# Autodesk Inventor assembly: Main Assembly
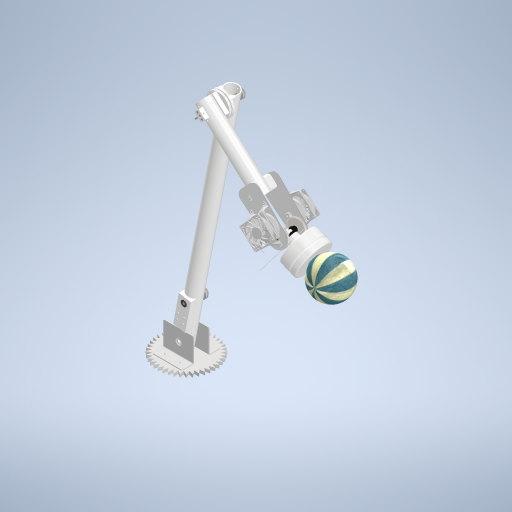
[picture p0: Inventor's stored thumbnail of the model, 512x512]
Saved by Autodesk Inventor 2023 (Build 270158000, 158)
## iProperties
Created: 2022-10-01
Part Number: Main Assembly
Document SubType Name: Assembly
Designer: cjj5381
Mass: 5668.97 g
Surface Area: 15277.1 cm^2
Volume: 4706.26 cm^3
Density: 1.20456 g/cm^3
Author: cjj5381
## Documents named in this file (24)
- C:\Users\t205b\OneDrive\Documents\Github\BehrendURCMechanical\CAD\Apparatus\THE ARM\Main Assembly.iam
- C:\Users\t205b\OneDrive\Documents\Github\BehrendURCMechanical\CAD\Apparatus\THE ARM\Arm Segment 1.ipt
- C:\Users\t205b\OneDrive\Documents\Github\BehrendURCMechanical\CAD\Apparatus\THE ARM\3 Stage HD - CIM Sport.iam
- C:\Users\t205b\OneDrive\Documents\Github\BehrendURCMechanical\CAD\Apparatus\THE ARM\Arm Segment 2.ipt
- C:\Users\t205b\OneDrive\Documents\Github\BehrendURCMechanical\CAD\Apparatus\THE ARM\Wrist\Wrist.iam
- C:\Users\t205b\OneDrive\Documents\Github\BehrendURCMechanical\CAD\Apparatus\THE ARM\Versaball.iam
- C:\Users\t205b\OneDrive\Documents\Github\BehrendURCMechanical\CAD\Apparatus\THE ARM\Hardware\91290A224_NO THREADS_Alloy Steel Socket Head Screw.ipt
- C:\Users\t205b\OneDrive\Documents\Github\BehrendURCMechanical\CAD\Apparatus\THE ARM\Hub Plate.ipt
- C:\Users\t205b\OneDrive\Documents\Github\BehrendURCMechanical\CAD\Apparatus\THE ARM\Hardware\5909K15_Needle-Roller Thrust Bearing.ipt
- C:\Users\t205b\OneDrive\Documents\Github\BehrendURCMechanical\CAD\Apparatus\THE ARM\Hardware\5909K75_1 mm Thick Washer for 20 mm Shaft Diameter Needle-Roller Thrust Bearing.ipt
- C:\Users\t205b\OneDrive\Documents\Github\BehrendURCMechanical\CAD\Apparatus\THE ARM\Motor Mount.ipt
- C:\Users\t205b\OneDrive\Documents\Github\BehrendURCMechanical\CAD\Apparatus\THE ARM\Hardware\91251A342_NO THREADS_Black-Oxide Alloy Steel Socket Head Screw.ipt
- C:\Users\t205b\OneDrive\Documents\Github\BehrendURCMechanical\CAD\Apparatus\THE ARM\Hardware\1265K77_Rotary Shaft-longer.ipt
- C:\Users\t205b\OneDrive\Documents\Github\BehrendURCMechanical\CAD\Apparatus\THE ARM\Axial Holder.ipt
- C:\Users\t205b\OneDrive\Documents\Github\BehrendURCMechanical\CAD\Apparatus\THE ARM\Hardware\GPA60GT2060-B-NK10.iam
- C:\Users\t205b\OneDrive\Documents\Github\BehrendURCMechanical\CAD\Apparatus\THE ARM\Hardware\2349K412_Permanently Lubricated Ball Bearing.ipt
- C:\Users\t205b\OneDrive\Documents\Github\BehrendURCMechanical\CAD\Apparatus\THE ARM\Hardware\1265K77_Rotary Shaft short.ipt
- C:\Users\t205b\OneDrive\Documents\Github\BehrendURCMechanical\CAD\Apparatus\THE ARM\Base\Base.iam
- C:\Users\t205b\OneDrive\Documents\Github\BehrendURCMechanical\CAD\Apparatus\THE ARM\Hardware\94645A102_NO THREADS_High-Strength Steel Nylon-Insert Locknut.ipt
- C:\Users\t205b\OneDrive\Documents\Github\BehrendURCMechanical\CAD\Apparatus\THE ARM\Hardware\94180A361_NO THREADS_Tapered Heat-Set Inserts for Plastic.ipt
- C:\Users\t205b\OneDrive\Documents\Github\BehrendURCMechanical\CAD\Apparatus\THE ARM\Hardware\91290A252_NO THREADS_Alloy Steel Socket Head Screw.ipt
- C:\Users\t205b\OneDrive\Documents\Github\BehrendURCMechanical\CAD\Apparatus\THE ARM\Hardware\91290A195_Black-Oxide Alloy Steel Socket Head Screw.ipt
- C:\Users\t205b\OneDrive\Documents\Github\BehrendURCMechanical\CAD\Apparatus\THE ARM\Hardware\91290A195_Black-Oxide Alloy Steel Socket Head Screw_CPY.ipt
- C:\Users\t205b\OneDrive\Documents\Github\BehrendURCMechanical\CAD\Apparatus\THE ARM\Hardware\1265K17_Rotary Shaft.ipt
## Components (45 placed, 23 different names)
1. Base:1 [sub-assembly] — Mate:1, Flush:1, Mate:2, Mate:3
2. Arm Segment 1:1 — Mate:2, Mate:3, Mate:4, Mate:5, Mate:12, Mate:13, Mate:48, Mate:49, Mate:50, Mate:51
3. 3 Stage HD - CIM Sport:2 [sub-assembly]
4. Arm Segment 2:1 — Mate:20, Mate:21, Mate:22, Mate:23, Mate:44, Mate:45, Mate:46, Mate:47, Mate:52, Flush:11
5. Wrist:1 [sub-assembly] — Mate:52, Flush:11, Mate:54, Mate:55, Mate:56, Mate:57, Mate:58, Mate:59, Mate:60, Mate:61, Mate:62, Mate:63
6. Versaball:1 [sub-assembly] — Mate:54, Mate:55, Mate:68
7. Hub Plate:1 — Mate:18, Mate:19, Mate:20, Mate:21, Mate:39, Mate:40, Mate:41, Flush:8
8. Hub Plate:2 — Mate:12, Mate:13, Mate:16, Mate:17, Mate:18, Mate:42, Flush:9, Mate:43, Flush:10
9. 5909K15_Needle-Roller Thrust Bearing:1 — Mate:14, Tangent:1, Tangent:2, Mate:15
10. 5909K75_1 mm Thick Washer for 20 mm Shaft Diameter Needle-Roller Thrust Bearing:1 — Mate:14, Tangent:1, Mate:17
11. 5909K75_1 mm Thick Washer for 20 mm Shaft Diameter Needle-Roller Thrust Bearing:2 — Tangent:2, Mate:15, Mate:16, Mate:19
12. Motor Mount:1 — Mate:4, Mate:5, Mate:6, Mate:7, Mate:8, Flush:2, Mate:9
13. 1265K77_Rotary Shaft-longer:1 — Mate:24, Mate:25, Mate:28, Flush:5
14. Axial Holder:1 — Mate:22, Mate:23, Mate:24, Mate:25
15. 91290A252_NO THREADS_Alloy Steel Socket Head Screw:1
16. GPA60GT2060-B-NK10:1 [sub-assembly] — Mate:28, Flush:5
17. GPA60GT2060-B-NK10:2 [sub-assembly] — Mate:11, Flush:4
18. 2349K412_Permanently Lubricated Ball Bearing:1 — Flush:2, Mate:9, Mate:10, Flush:3
19. 1265K77_Rotary Shaft short:1 — Mate:10, Flush:3, Mate:11, Flush:4
20. 3 Stage HD - CIM Sport:3 [sub-assembly]
21. 91290A252_NO THREADS_Alloy Steel Socket Head Screw:2
22. 91290A252_NO THREADS_Alloy Steel Socket Head Screw:3
23. 94645A102_NO THREADS_High-Strength Steel Nylon-Insert Locknut:1
24. 94645A102_NO THREADS_High-Strength Steel Nylon-Insert Locknut:2
25. 94180A361_NO THREADS_Tapered Heat-Set Inserts for Plastic:1 — Mate:39, Mate:40
26. 94180A361_NO THREADS_Tapered Heat-Set Inserts for Plastic:2 — Mate:41, Flush:8
27. 94180A361_NO THREADS_Tapered Heat-Set Inserts for Plastic:3 — Mate:43, Flush:10
28. 94180A361_NO THREADS_Tapered Heat-Set Inserts for Plastic:4 — Mate:42, Flush:9
29. 91290A224_NO THREADS_Alloy Steel Socket Head Screw:7 — Mate:44, Mate:45
30. 91290A224_NO THREADS_Alloy Steel Socket Head Screw:8 — Mate:46, Mate:47
31. 91290A224_NO THREADS_Alloy Steel Socket Head Screw:9 — Mate:50, Mate:51
32. 91290A224_NO THREADS_Alloy Steel Socket Head Screw:10 — Mate:48, Mate:49
33. 91290A195_Black-Oxide Alloy Steel Socket Head Screw:1 — Mate:56, Mate:57, Mate:66, Flush:13
34. 91290A195_Black-Oxide Alloy Steel Socket Head Screw_CPY:1 — Mate:58, Mate:59, Mate:67, Flush:14
35. 91290A195_Black-Oxide Alloy Steel Socket Head Screw:2 — Mate:60, Mate:61, Mate:64, Flush:15
36. 91290A195_Black-Oxide Alloy Steel Socket Head Screw:3 — Mate:62, Mate:63, Mate:65, Flush:12
37. 94645A102_NO THREADS_High-Strength Steel Nylon-Insert Locknut:3 — Mate:64, Flush:15
38. 94645A102_NO THREADS_High-Strength Steel Nylon-Insert Locknut:4 — Mate:65, Flush:12
39. 94645A102_NO THREADS_High-Strength Steel Nylon-Insert Locknut:5 — Mate:67, Flush:14
40. 94645A102_NO THREADS_High-Strength Steel Nylon-Insert Locknut:6 — Mate:66, Flush:13
41. 1265K17_Rotary Shaft:1 — Mate:68
42. 91251A342_NO THREADS_Black-Oxide Alloy Steel Socket Head Screw:1 — Mate:6
43. 91251A342_NO THREADS_Black-Oxide Alloy Steel Socket Head Screw:2 — Mate:7, Mate:8
44. 91251A342_NO THREADS_Black-Oxide Alloy Steel Socket Head Screw:3
45. 91251A342_NO THREADS_Black-Oxide Alloy Steel Socket Head Screw:4
## Component patterns: (4 elements, first: 91251A342_NO THREADS_Black-Oxide Alloy Steel Socket Head Screw:1)
## Relationships (80: Mate 63, Flush 15, Tangent 2)
- Mate:1: Base:1
- Flush:1: Base:1
- Mate:2: Base:1 ↔ Arm Segment 1:1
- Mate:3: Base:1 ↔ Arm Segment 1:1
- Mate:4: Arm Segment 1:1 ↔ Motor Mount:1
- Mate:5: Arm Segment 1:1 ↔ Motor Mount:1
- Mate:6: Motor Mount:1 ↔ 91251A342_NO THREADS_Black-Oxide Alloy Steel Socket Head Screw:1
- Mate:7: Motor Mount:1 ↔ 91251A342_NO THREADS_Black-Oxide Alloy Steel Socket Head Screw:2
- Mate:8: Motor Mount:1 ↔ 91251A342_NO THREADS_Black-Oxide Alloy Steel Socket Head Screw:2
- Flush:2: Motor Mount:1 ↔ 2349K412_Permanently Lubricated Ball Bearing:1
- Mate:9: Motor Mount:1 ↔ 2349K412_Permanently Lubricated Ball Bearing:1
- Mate:10: 2349K412_Permanently Lubricated Ball Bearing:1 ↔ 1265K77_Rotary Shaft short:1
- Flush:3: 2349K412_Permanently Lubricated Ball Bearing:1 ↔ 1265K77_Rotary Shaft short:1
- Mate:11: GPA60GT2060-B-NK10:2 ↔ 1265K77_Rotary Shaft short:1
- Flush:4: GPA60GT2060-B-NK10:2 ↔ 1265K77_Rotary Shaft short:1
- Mate:12: Arm Segment 1:1 ↔ Hub Plate:2
- Mate:13: Arm Segment 1:1 ↔ Hub Plate:2
- Mate:14: 5909K15_Needle-Roller Thrust Bearing:1 ↔ 5909K75_1 mm Thick Washer for 20 mm Shaft Diameter Needle-Roller Thrust Bearing:1
- Tangent:1: 5909K15_Needle-Roller Thrust Bearing:1 ↔ 5909K75_1 mm Thick Washer for 20 mm Shaft Diameter Needle-Roller Thrust Bearing:1
- Tangent:2: 5909K15_Needle-Roller Thrust Bearing:1 ↔ 5909K75_1 mm Thick Washer for 20 mm Shaft Diameter Needle-Roller Thrust Bearing:2
- Mate:15: 5909K15_Needle-Roller Thrust Bearing:1 ↔ 5909K75_1 mm Thick Washer for 20 mm Shaft Diameter Needle-Roller Thrust Bearing:2
- Mate:16: Hub Plate:2 ↔ 5909K75_1 mm Thick Washer for 20 mm Shaft Diameter Needle-Roller Thrust Bearing:2
- Mate:17: Hub Plate:2 ↔ 5909K75_1 mm Thick Washer for 20 mm Shaft Diameter Needle-Roller Thrust Bearing:1
- Mate:18: Hub Plate:1 ↔ Hub Plate:2
- Mate:19: Hub Plate:1 ↔ 5909K75_1 mm Thick Washer for 20 mm Shaft Diameter Needle-Roller Thrust Bearing:2
- Mate:20: Arm Segment 2:1 ↔ Hub Plate:1
- Mate:21: Arm Segment 2:1 ↔ Hub Plate:1
- Mate:22: Arm Segment 2:1 ↔ Axial Holder:1
- Mate:23: Arm Segment 2:1 ↔ Axial Holder:1
- Mate:24: 1265K77_Rotary Shaft-longer:1 ↔ Axial Holder:1
- Mate:25: 1265K77_Rotary Shaft-longer:1 ↔ Axial Holder:1
- [Mate]: Axial Holder:1 ↔ 91290A252_NO THREADS_Alloy Steel Socket Head Screw:1
- [Mate]: Axial Holder:1 ↔ 91290A252_NO THREADS_Alloy Steel Socket Head Screw:1
- Mate:28: 1265K77_Rotary Shaft-longer:1 ↔ GPA60GT2060-B-NK10:1
- Flush:5: 1265K77_Rotary Shaft-longer:1 ↔ GPA60GT2060-B-NK10:1
- [Mate]: Axial Holder:1 ↔ 91290A252_NO THREADS_Alloy Steel Socket Head Screw:2
- [Mate]: Axial Holder:1 ↔ 91290A252_NO THREADS_Alloy Steel Socket Head Screw:2
- [Mate]: Axial Holder:1 ↔ 91290A252_NO THREADS_Alloy Steel Socket Head Screw:3
- [Mate]: Axial Holder:1 ↔ 91290A252_NO THREADS_Alloy Steel Socket Head Screw:3
- [Mate]: 91290A252_NO THREADS_Alloy Steel Socket Head Screw:2 ↔ 94645A102_NO THREADS_High-Strength Steel Nylon-Insert Locknut:1
- [Flush]: 91290A252_NO THREADS_Alloy Steel Socket Head Screw:2 ↔ 94645A102_NO THREADS_High-Strength Steel Nylon-Insert Locknut:1
- [Mate]: 91290A252_NO THREADS_Alloy Steel Socket Head Screw:3 ↔ 94645A102_NO THREADS_High-Strength Steel Nylon-Insert Locknut:2
- [Flush]: 91290A252_NO THREADS_Alloy Steel Socket Head Screw:3 ↔ 94645A102_NO THREADS_High-Strength Steel Nylon-Insert Locknut:2
- Mate:39: Hub Plate:1 ↔ 94180A361_NO THREADS_Tapered Heat-Set Inserts for Plastic:1
- Mate:40 (1 mm): Hub Plate:1 ↔ 94180A361_NO THREADS_Tapered Heat-Set Inserts for Plastic:1
- Mate:41: Hub Plate:1 ↔ 94180A361_NO THREADS_Tapered Heat-Set Inserts for Plastic:2
- Flush:8 (-1 mm): Hub Plate:1 ↔ 94180A361_NO THREADS_Tapered Heat-Set Inserts for Plastic:2
- Mate:42: Hub Plate:2 ↔ 94180A361_NO THREADS_Tapered Heat-Set Inserts for Plastic:4
- Flush:9 (-1 mm): Hub Plate:2 ↔ 94180A361_NO THREADS_Tapered Heat-Set Inserts for Plastic:4
- Mate:43: Hub Plate:2 ↔ 94180A361_NO THREADS_Tapered Heat-Set Inserts for Plastic:3
- Flush:10 (-1 mm): Hub Plate:2 ↔ 94180A361_NO THREADS_Tapered Heat-Set Inserts for Plastic:3
- Mate:44: Arm Segment 2:1 ↔ 91290A224_NO THREADS_Alloy Steel Socket Head Screw:7
- Mate:45 (-25.5 mm): Arm Segment 2:1 ↔ 91290A224_NO THREADS_Alloy Steel Socket Head Screw:7
- Mate:46: Arm Segment 2:1 ↔ 91290A224_NO THREADS_Alloy Steel Socket Head Screw:8
- Mate:47 (-25.5 mm): Arm Segment 2:1 ↔ 91290A224_NO THREADS_Alloy Steel Socket Head Screw:8
- Mate:48: Arm Segment 1:1 ↔ 91290A224_NO THREADS_Alloy Steel Socket Head Screw:10
- Mate:49 (-25.5 mm): Arm Segment 1:1 ↔ 91290A224_NO THREADS_Alloy Steel Socket Head Screw:10
- Mate:50: Arm Segment 1:1 ↔ 91290A224_NO THREADS_Alloy Steel Socket Head Screw:9
- Mate:51 (-25.5 mm): Arm Segment 1:1 ↔ 91290A224_NO THREADS_Alloy Steel Socket Head Screw:9
- Mate:52: Arm Segment 2:1 ↔ Wrist:1
- Flush:11: Arm Segment 2:1 ↔ Wrist:1
- Mate:54: Wrist:1 ↔ Versaball:1
- Mate:55: Wrist:1 ↔ Versaball:1
- Mate:56: Wrist:1 ↔ 91290A195_Black-Oxide Alloy Steel Socket Head Screw:1
- Mate:57: Wrist:1 ↔ 91290A195_Black-Oxide Alloy Steel Socket Head Screw:1
- Mate:58: Wrist:1 ↔ 91290A195_Black-Oxide Alloy Steel Socket Head Screw_CPY:1
- Mate:59: Wrist:1 ↔ 91290A195_Black-Oxide Alloy Steel Socket Head Screw_CPY:1
- Mate:60: Wrist:1 ↔ 91290A195_Black-Oxide Alloy Steel Socket Head Screw:2
- Mate:61: Wrist:1 ↔ 91290A195_Black-Oxide Alloy Steel Socket Head Screw:2
- Mate:62: Wrist:1 ↔ 91290A195_Black-Oxide Alloy Steel Socket Head Screw:3
- Mate:63: Wrist:1 ↔ 91290A195_Black-Oxide Alloy Steel Socket Head Screw:3
- Mate:64: 91290A195_Black-Oxide Alloy Steel Socket Head Screw:2 ↔ 94645A102_NO THREADS_High-Strength Steel Nylon-Insert Locknut:3
- Mate:65: 91290A195_Black-Oxide Alloy Steel Socket Head Screw:3 ↔ 94645A102_NO THREADS_High-Strength Steel Nylon-Insert Locknut:4
- Flush:12: 91290A195_Black-Oxide Alloy Steel Socket Head Screw:3 ↔ 94645A102_NO THREADS_High-Strength Steel Nylon-Insert Locknut:4
- Mate:66: 91290A195_Black-Oxide Alloy Steel Socket Head Screw:1 ↔ 94645A102_NO THREADS_High-Strength Steel Nylon-Insert Locknut:6
- Flush:13: 91290A195_Black-Oxide Alloy Steel Socket Head Screw:1 ↔ 94645A102_NO THREADS_High-Strength Steel Nylon-Insert Locknut:6
- Mate:67: 91290A195_Black-Oxide Alloy Steel Socket Head Screw_CPY:1 ↔ 94645A102_NO THREADS_High-Strength Steel Nylon-Insert Locknut:5
- Flush:14: 91290A195_Black-Oxide Alloy Steel Socket Head Screw_CPY:1 ↔ 94645A102_NO THREADS_High-Strength Steel Nylon-Insert Locknut:5
- Mate:68: Versaball:1 ↔ 1265K17_Rotary Shaft:1
- Flush:15: 91290A195_Black-Oxide Alloy Steel Socket Head Screw:2 ↔ 94645A102_NO THREADS_High-Strength Steel Nylon-Insert Locknut:3
